# Autodesk Inventor assembly: Michelson_assembly
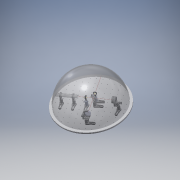
[picture p0: Inventor's stored thumbnail of the model, 180x180]
Saved by Autodesk Inventor 2016 (Build 200138000, 138)
## iProperties
Created: 2016-01-13
Part Number: Michelson_assembly
Document SubType Name: Assembly
Designer: Conor Mow-Lowry
Mass: 14949.3 g
Surface Area: 21194.6 cm^2
Volume: 6974.17 cm^3
Density: 2.14353 g/cm^3
Author: Conor Mow-Lowry
## Documents named in this file (15)
- C:\Documents\Birmingham\Outreach\ThinkTank Michelson\Michelson_assembly.iam
- C:\Documents\Birmingham\Outreach\ThinkTank Michelson\Circular_Breadboard.ipt
- C:\Documents\Birmingham\Outreach\ThinkTank Michelson\newport_sn200-f2k.ipt
- C:\Documents\Birmingham\Outreach\ThinkTank Michelson\Mirror 2 inch.ipt
- C:\Documents\Birmingham\Outreach\ThinkTank Michelson\PZTMirrorAssembly.iam
- C:\Documents\Birmingham\Outreach\ThinkTank Michelson\BSholder.ipt
- C:\Documents\Birmingham\Outreach\ThinkTank Michelson\Beamsplitter 2 inch.ipt
- C:\Documents\Birmingham\Outreach\ThinkTank Michelson\RS2P4M-Step.ipt
- C:\Documents\Birmingham\Outreach\ThinkTank Michelson\Laser_Assembly.iam
- C:\Documents\Birmingham\Outreach\ThinkTank Michelson\beam small 100.ipt
- C:\Documents\Birmingham\Outreach\ThinkTank Michelson\Dome.ipt
- C:\Documents\Birmingham\Outreach\ThinkTank Michelson\beam small 101.ipt
- C:\Documents\Birmingham\Outreach\ThinkTank Michelson\CF125-Step.ipt
- C:\Documents\Birmingham\Outreach\ThinkTank Michelson\beam small 102.ipt
- C:\Documents\Birmingham\Outreach\ThinkTank Michelson\Lens_mounted.iam
## Components (24 placed, 14 different names)
1. Circular_Breadboard:1 — Mate:20, Mate:23, Mate:24, Mate:25, Flush:1, Mate:31, Angle:3, Angle:4, Angle:5, Angle:6, Mate:37, Mate:38, Mate:39, Mate:40, Mate:41, Angle:7, Angle:8, Mate:51, Mate:52
2. RS2P4M-Step:1 — Mate:46
3. RS2P4M-Step:3 — Angle:1, Mate:45
4. RS2P4M-Step:4 — Mate:44
5. newport_sn200-f2k:1 — Mate:12, Mate:13
6. newport_sn200-f2k:2 — Mate:14, Mate:15
7. Mirror 2 inch:1 — Mate:12, Mate:13, Angle:4, Mate:34, Mate:57
8. PZTMirrorAssembly:1 [sub-assembly] — Mate:14, Mate:15, Mate:35, Angle:5, Mate:55, Mate:56
9. BSholder:1 — Mate:19, Mate:27
10. Beamsplitter 2 inch:1 — Mate:19, Mate:27, Angle:1, Mate:32, Angle:6, Mate:36, Mate:49
11. Laser_Assembly:1 [sub-assembly] — Mate:20, Mate:21, Mate:22, Mate:23, Flush:1, Mate:42, Mate:43
12. beam small 100:1 — Mate:21, Mate:22, Mate:32, Mate:35, Mate:47, Mate:55
13. Dome:1 — Mate:24, Mate:25
14. beam small 101:1 — Mate:31, Angle:3, Mate:34, Mate:36, Mate:48, Mate:56, Mate:57
15. CF125-Step:1 — Mate:37, Mate:44
16. CF125-Step:2 — Mate:38, Mate:45
17. CF125-Step:3 — Mate:39, Mate:46
18. CF125-Step:4 — Mate:40, Mate:43
19. CF125-Step:5 — Mate:41, Mate:42
20. beam small 102:1 — Mate:48, Mate:49, Mate:50
21. Lens_mounted:1 [sub-assembly] — Mate:47, Angle:7, Mate:53
22. Lens_mounted:2 [sub-assembly] — Mate:50, Angle:8, Mate:54
23. CF125-Step:6 — Mate:51, Mate:53
24. CF125-Step:7 — Mate:52, Mate:54
## Relationships (55: Mate 47, Angle 7, Flush 1)
- [Mate]: Circular_Breadboard:1 ↔ RS2P4M-Step:4
- [Mate]: Circular_Breadboard:1 ↔ RS2P4M-Step:1
- [Mate]: Circular_Breadboard:1 ↔ RS2P4M-Step:3
- [Mate]: RS2P4M-Step:1 ↔ newport_sn200-f2k:2
- [Mate]: RS2P4M-Step:4 ↔ newport_sn200-f2k:1
- [Mate]: RS2P4M-Step:4 ↔ newport_sn200-f2k:1
- [Mate]: RS2P4M-Step:1 ↔ newport_sn200-f2k:2
- Mate:12: newport_sn200-f2k:1 ↔ Mirror 2 inch:1
- Mate:13: newport_sn200-f2k:1 ↔ Mirror 2 inch:1
- Mate:14: newport_sn200-f2k:2 ↔ PZTMirrorAssembly:1
- Mate:15: newport_sn200-f2k:2 ↔ PZTMirrorAssembly:1
- [Mate]: RS2P4M-Step:3 ↔ BSholder:1
- [Mate]: RS2P4M-Step:3 ↔ BSholder:1
- Mate:19: BSholder:1 ↔ Beamsplitter 2 inch:1
- Mate:20: Circular_Breadboard:1 ↔ Laser_Assembly:1
- Mate:21: Laser_Assembly:1 ↔ beam small 100:1
- Mate:22: Laser_Assembly:1 ↔ beam small 100:1
- Mate:23 (25 mm): Circular_Breadboard:1 ↔ Laser_Assembly:1
- Mate:24: Circular_Breadboard:1 ↔ Dome:1
- Mate:25: Circular_Breadboard:1 ↔ Dome:1
- Flush:1 (85 mm): Circular_Breadboard:1 ↔ Laser_Assembly:1
- Mate:27: BSholder:1 ↔ Beamsplitter 2 inch:1
- Mate:31 (88.1 mm): Circular_Breadboard:1 ↔ beam small 101:1
- Angle:1 (0 deg): RS2P4M-Step:3 ↔ Beamsplitter 2 inch:1
- Mate:32: Beamsplitter 2 inch:1 ↔ beam small 100:1
- Angle:3 (0 deg): Circular_Breadboard:1 ↔ beam small 101:1
- Angle:4 (180 deg): Circular_Breadboard:1 ↔ Mirror 2 inch:1
- Mate:34: Mirror 2 inch:1 ↔ beam small 101:1
- Mate:35: PZTMirrorAssembly:1 ↔ beam small 100:1
- Angle:5 (0 deg): Circular_Breadboard:1 ↔ PZTMirrorAssembly:1
- Angle:6 (135 deg): Circular_Breadboard:1 ↔ Beamsplitter 2 inch:1
- Mate:36: Beamsplitter 2 inch:1 ↔ beam small 101:1
- Mate:37: Circular_Breadboard:1 ↔ CF125-Step:1
- Mate:38: Circular_Breadboard:1 ↔ CF125-Step:2
- Mate:39: Circular_Breadboard:1 ↔ CF125-Step:3
- Mate:40: Circular_Breadboard:1 ↔ CF125-Step:4
- Mate:41: Circular_Breadboard:1 ↔ CF125-Step:5
- Mate:42: Laser_Assembly:1 ↔ CF125-Step:5
- Mate:43: Laser_Assembly:1 ↔ CF125-Step:4
- Mate:44: RS2P4M-Step:4 ↔ CF125-Step:1
- Mate:45: RS2P4M-Step:3 ↔ CF125-Step:2
- Mate:46: RS2P4M-Step:1 ↔ CF125-Step:3
- Mate:47: beam small 100:1 ↔ Lens_mounted:1
- Angle:7 (180 deg): Circular_Breadboard:1 ↔ Lens_mounted:1
- Mate:48: beam small 101:1 ↔ beam small 102:1
- Mate:49: Beamsplitter 2 inch:1 ↔ beam small 102:1
- Mate:50: beam small 102:1 ↔ Lens_mounted:2
- Angle:8 (180 deg): Circular_Breadboard:1 ↔ Lens_mounted:2
- Mate:51: Circular_Breadboard:1 ↔ CF125-Step:6
- Mate:52: Circular_Breadboard:1 ↔ CF125-Step:7
- Mate:53: Lens_mounted:1 ↔ CF125-Step:6
- Mate:54: Lens_mounted:2 ↔ CF125-Step:7
- Mate:55: PZTMirrorAssembly:1 ↔ beam small 100:1
- Mate:56 (150 mm): PZTMirrorAssembly:1 ↔ beam small 101:1
- Mate:57: Mirror 2 inch:1 ↔ beam small 101:1
